# Autodesk Inventor assembly: Aufhängung_Version2
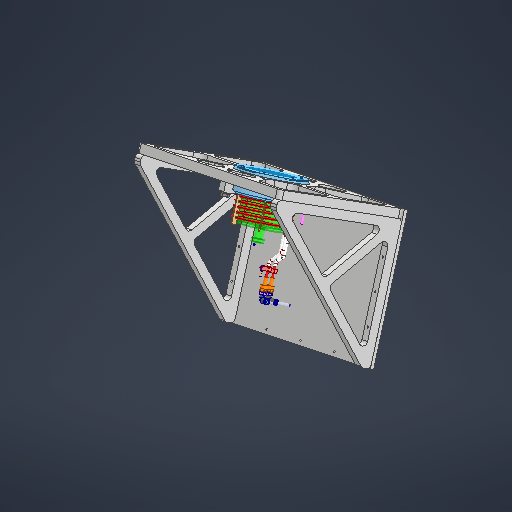
[picture p0: Inventor's stored thumbnail of the model, 512x512]
Saved by Autodesk Inventor 2027 (Build 310192060, 192F)
## iProperties
Created: 2026-07-21
Part Number: Aufhängung_Version2
Document SubType Name: Assembly
Designer: kw
Author: kw
## Documents named in this file (6)
- C:\Users\kw\OneDrive\Documents\Uni\Masterthesis\Spezialisierungsmodul\InventorZeichnungen\Koppeltest_Halterung\Aufhängung_RIT10.iam
- C:\Users\kw\OneDrive\Documents\Uni\Masterthesis\Spezialisierungsmodul\InventorZeichnungen\Koppeltest_Halterung\Aufhängung_Seitenteil.ipt
- C:\Users\kw\OneDrive\Documents\Uni\Masterthesis\Spezialisierungsmodul\InventorZeichnungen\Koppeltest_Halterung\Halterung_Teflonplatte.ipt
- C:\Users\kw\OneDrive\Documents\Uni\Masterthesis\Spezialisierungsmodul\InventorZeichnungen\Koppeltest_Halterung\Pratze_ISO-K160.ipt
- C:\Users\kw\OneDrive\Documents\Uni\Masterthesis\Spezialisierungsmodul\InventorZeichnungen\Koppeltest_Halterung\Aufhängung_Front_RIT10.ipt
- C:\Users\kw\OneDrive\Documents\Uni\Masterthesis\Spezialisierungsmodul\InventorZeichnungen\19K_001_010_00_A_RIM_10_2019_EFRE_3D_2024_0228\19K_001_010_00_A_RIM_10_2019_EFRE_3D_2024_0228.ipt
## Components (6 placed, 5 different names)
1. Aufhängung_Seitenteil:1 — Mate:1, Flush:1, Flush:2
2. Halterung_Teflonplatte:1 — Mate:1, Flush:1, Flush:2, Mate:2, Flush:3, Flush:4, Mate:3, Flush:5, Flush:6
3. Aufhängung_Seitenteil:2 — Mate:2, Flush:3, Flush:4
4. Pratze_ISO-K160:4 — Mate:7, Flush:7
5. Aufhängung_Front_RIT10:1 — Mate:3, Flush:5, Flush:6, Mate:5, Mate:6, Mate:7, Flush:7
6. 19K_001_010_00_A_RIM_10_2019_EFRE_3D_2024_0228:1 — Mate:5, Mate:6
## Relationships (13: Flush 7, Mate 6)
- Mate:1: Aufhängung_Seitenteil:1 ↔ Halterung_Teflonplatte:1
- Flush:1: Aufhängung_Seitenteil:1 ↔ Halterung_Teflonplatte:1
- Flush:2 (20 mm): Aufhängung_Seitenteil:1 ↔ Halterung_Teflonplatte:1
- Mate:2: Halterung_Teflonplatte:1 ↔ Aufhängung_Seitenteil:2
- Flush:3: Halterung_Teflonplatte:1 ↔ Aufhängung_Seitenteil:2
- Flush:4 (20 mm): Halterung_Teflonplatte:1 ↔ Aufhängung_Seitenteil:2
- Mate:3: Halterung_Teflonplatte:1 ↔ Aufhängung_Front_RIT10:1
- Flush:5: Halterung_Teflonplatte:1 ↔ Aufhängung_Front_RIT10:1
- Flush:6: Halterung_Teflonplatte:1 ↔ Aufhängung_Front_RIT10:1
- Mate:5: Aufhängung_Front_RIT10:1 ↔ 19K_001_010_00_A_RIM_10_2019_EFRE_3D_2024_0228:1
- Mate:6: Aufhängung_Front_RIT10:1 ↔ 19K_001_010_00_A_RIM_10_2019_EFRE_3D_2024_0228:1
- Mate:7: Pratze_ISO-K160:4 ↔ Aufhängung_Front_RIT10:1
- Flush:7 (39.95 mm): Pratze_ISO-K160:4 ↔ Aufhängung_Front_RIT10:1
